# Autodesk Inventor assembly: 6P 24T Sprocket, No Insert_mirrored
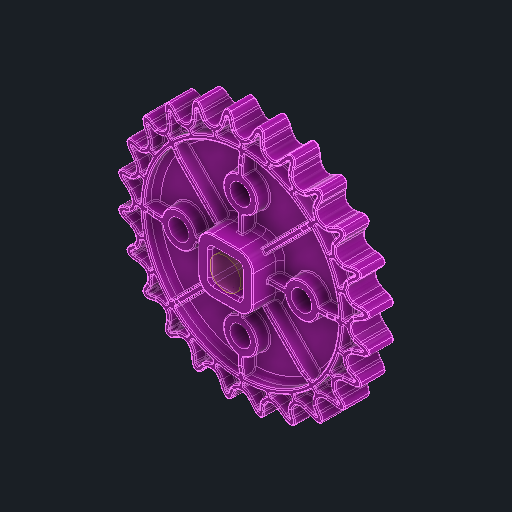
[picture p0: Inventor's stored thumbnail of the model, 512x512]
Saved by Autodesk Inventor 2024 (Build 280153000, 153)
## iProperties
Created: 2022-08-02
Part Number: 6P 24T Sprocket, No Insert_mirrored
Document SubType Name: Assembly
Designer: Averey Ku
Author: ylu12
## Documents named in this file (2)
- D:\vex_robotics\hardware\cad\lil_zoom\intake\mirrored_parts\6P 24T Sprocket, No Insert_mirrored.iam
- D:\vex_robotics\hardware\cad\lil_zoom\intake\mirrored_parts\6P 24T Sprocket_mirrored.ipt
## Components (1 placed, 1 different names)
1. 6P 24T Sprocket_mirrored:1 — Mate:10, Mate:9, Flush:5
## Relationships (3: Mate 2, Flush 1)
- Mate:10: 6P 24T Sprocket_mirrored:1
- Mate:9: 6P 24T Sprocket_mirrored:1
- Flush:5: 6P 24T Sprocket_mirrored:1
